# Autodesk Inventor assembly: 0008-10-03 YAxis
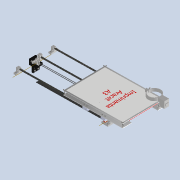
[picture p0: Inventor's stored thumbnail of the model, 180x180]
Saved by Autodesk Inventor 2020 (Build 240168000, 168)
## iProperties
Created: 2021-02-20
Part Number: 0008-10-03 YAxis
Document SubType Name: Assembly
Designer: Iulian Bors
Description: Y axis
Author: Iulian Bors
Subject: 10-03
## Documents named in this file (39)
- Z:\I.A.B\Proiecte\0008 I.A.B 3D 2.1 Imprimanta aracet Metal\10 Mecanic\0008-10-03 YAxis.iam
- Z:\I.A.B\Proiecte\0008 I.A.B 3D 2.1 Imprimanta aracet Metal\10 Mecanic\Foaie A3.ipt
- Z:\I.A.B\Proiecte\0008 I.A.B 3D 2.1 Imprimanta aracet Metal\10 Mecanic\0008-10-1001 NEMA17 - Motor de passo.ipt
- Z:\I.A.B\Proiecte\0008 I.A.B 3D 2.1 Imprimanta aracet Metal\10 Mecanic\0008-10-1011 GT2 Timing Pulley 20 Tooth.ipt
- Z:\I.A.B\Proiecte\0008 I.A.B 3D 2.1 Imprimanta aracet Metal\10 Mecanic\0008-10-1012 16T W6 B3 Without T_Shrinkwrap_1.ipt
- Z:\I.A.B\Proiecte\0008 I.A.B 3D 2.1 Imprimanta aracet Metal\10 Mecanic\0008-10-017 Heated bed.ipt
- Z:\I.A.B\Proiecte\0008 I.A.B 3D 2.1 Imprimanta aracet Metal\10 Mecanic\0008-10-018 Suport Heated Bed.ipt
- Z:\I.A.B\Proiecte\0008 I.A.B 3D 2.1 Imprimanta aracet Metal\10 Mecanic\0008-10-1016 SC10UU.ipt
- Z:\I.A.B\Proiecte\0008 I.A.B 3D 2.1 Imprimanta aracet Metal\10 Mecanic\0008-10-1017 Bara 10.ipt
- Z:\I.A.B\Proiecte\0008 I.A.B 3D 2.1 Imprimanta aracet Metal\10 Mecanic\0008-10-019 Suport Axa Y.ipt
- Z:\I.A.B\Proiecte\0008 I.A.B 3D 2.1 Imprimanta aracet Metal\10 Mecanic\0008-10-020 Suport Axa Y.ipt
- Z:\I.A.B\Proiecte\0008 I.A.B 3D 2.1 Imprimanta aracet Metal\10 Mecanic\0008-10-037.ipt
- Z:\I.A.B\Proiecte\0008 I.A.B 3D 2.1 Imprimanta aracet Metal\10 Mecanic\0008-10-036.ipt
- Z:\I.A.B\Proiecte\0008 I.A.B 3D 2.1 Imprimanta aracet Metal\20 Electric\0008-20-1003 Switch.ipt
- Z:\I.A.B\Proiecte\0008 I.A.B 3D 2.1 Imprimanta aracet Metal\10 Mecanic\0008-10-047 Suport Rulment Sc si curea.ipt
- Z:\I.A.B\Proiecte\0008 I.A.B 3D 2.1 Imprimanta aracet Metal\10 Mecanic\0008-10-048.ipt
- Z:\I.A.B\Proiecte\0008 I.A.B 3D 2.1 Imprimanta aracet Metal\10 Mecanic\0008-10-052 Suport Axa Y +Senzor.ipt
- Z:\I.A.B\Proiecte\0008 I.A.B 3D 2.1 Imprimanta aracet Metal\10 Mecanic\0008-10-054 Suport doking.ipt
- Z:\I.A.B\Proiecte\0008 I.A.B 3D 2.1 Imprimanta aracet Metal\10 Mecanic\0008-10-2016 DIN 315 - M4.ipt
- Z:\I.A.B\Proiecte\0008 I.A.B 3D 2.1 Imprimanta aracet Metal\10 Mecanic\0008-10-2017 DIN 7991 - M4x20.ipt
- Z:\I.A.B\Proiecte\0008 I.A.B 3D 2.1 Imprimanta aracet Metal\10 Mecanic\0008-10-055 Doking.ipt
- Z:\I.A.B\Proiecte\0008 I.A.B 3D 2.1 Imprimanta aracet Metal\10 Mecanic\0008-10-2000 DIN 6912 - M4 x 25.ipt
- Z:\I.A.B\Proiecte\0008 I.A.B 3D 2.1 Imprimanta aracet Metal\20 Electric\0008-20-1007 HEATING BED.ipt
- Z:\I.A.B\Proiecte\0008 I.A.B 3D 2.1 Imprimanta aracet Metal\10 Mecanic\0008-10-01 Sckeleton_Shrinkwrap.ipt
- Z:\I.A.B\Proiecte\0008 I.A.B 3D 2.1 Imprimanta aracet Metal\10 Mecanic\0008-10-2002 DIN 125 - A 4.3.ipt
- Z:\I.A.B\Proiecte\0008 I.A.B 3D 2.1 Imprimanta aracet Metal\10 Mecanic\0008-10-2010 M 5 Canal.ipt
- Z:\I.A.B\Proiecte\0008 I.A.B 3D 2.1 Imprimanta aracet Metal\10 Mecanic\0008-10-2011 DIN 7984 - M5 x 16.ipt
- Z:\I.A.B\Proiecte\0008 I.A.B 3D 2.1 Imprimanta aracet Metal\10 Mecanic\0008-10-2012 DIN 125 - A 5.3.ipt
- Z:\I.A.B\Proiecte\0008 I.A.B 3D 2.1 Imprimanta aracet Metal\10 Mecanic\SurubM4x25.iam
- Z:\I.A.B\Proiecte\0008 I.A.B 3D 2.1 Imprimanta aracet Metal\10 Mecanic\0008-10-2005 DIN 125 - A 3.2.ipt
- Z:\I.A.B\Proiecte\0008 I.A.B 3D 2.1 Imprimanta aracet Metal\10 Mecanic\0008-10-2006 DIN 7984 - M3 x 16.ipt
- Z:\I.A.B\Proiecte\0008 I.A.B 3D 2.1 Imprimanta aracet Metal\10 Mecanic\0008-10-2018 DIN 912 - M4 x 0.7 x 40.ipt
- Z:\I.A.B\Proiecte\0008 I.A.B 3D 2.1 Imprimanta aracet Metal\10 Mecanic\0008-10-2001 DIN 934 - M4 x 0.7.ipt
- Z:\I.A.B\Proiecte\0008 I.A.B 3D 2.1 Imprimanta aracet Metal\10 Mecanic\0008-10-1023 Compress Spring11.ipt
- Z:\I.A.B\Proiecte\0008 I.A.B 3D 2.1 Imprimanta aracet Metal\10 Mecanic\0008-10-03 YAxis\Design Accelerator\Synchronous Belts Transmission1.iam
- Z:\I.A.B\Proiecte\0008 I.A.B 3D 2.1 Imprimanta aracet Metal\10 Mecanic\0008-10-1026 wire chain Y.ipt
- Z:\I.A.B\Proiecte\0008 I.A.B 3D 2.1 Imprimanta aracet Metal\10 Mecanic\0008-10-2024 DIN 7991 - M4  x  35.ipt
- Z:\I.A.B\Proiecte\0008 I.A.B 3D 2.1 Imprimanta aracet Metal\10 Mecanic\0008-10-2027 DIN 7984 - M3 x 5.ipt
- Z:\I.A.B\Proiecte\0008 I.A.B 3D 2.1 Imprimanta aracet Metal\10 Mecanic\0008-10-2040 DIN 7984 - M5 x 20.ipt
## Components (189 placed, 39 different names)
1. Foaie A3.ipt:1 — Mate:59, Flush:56, Flush:57, Angle:8, Mate:216
2. 0008-10-017 Heated bed.ipt:2 — Mate:59, Flush:56, Flush:57, Mate:60, Mate:61, Mate:62, Mate:213, Mate:214, Flush:141
3. 0008-10-018 Suport Heated Bed.ipt:3 — Mate:60, Mate:61, Mate:62, Mate:65, Flush:59, Mate:66, Flush:61, Mate:68, Mate:69, Flush:64, Flush:65, Angle:9, Mate:73, Mate:74, Mate:78, Mate:197, Insert:33, Insert:36, Angle:32, Insert:48, Insert:49, Insert:50, Insert:51, Insert:56, Insert:57, Insert:58, Insert:59, Insert:64, Insert:65, Insert:66, Insert:67, Insert:72, Insert:73, Insert:74, Insert:75, Insert:80, Insert:81, Insert:82, Insert:83, Insert:102, Insert:103, Insert:160, Insert:164, Insert:165, Insert:166, Mate:226, Insert:191
4. 0008-10-1016 SC10UU.ipt:4 — Mate:69, Flush:63, Flush:64, Mate:228
5. 0008-10-1016 SC10UU.ipt:5 — Mate:66, Mate:67, Flush:60, Flush:63
6. 0008-10-1016 SC10UU.ipt:6 — Mate:68, Flush:62, Flush:65, Mate:70
7. 0008-10-1016 SC10UU.ipt:7 — Mate:65, Flush:59, Mate:67, Flush:60, Flush:61, Flush:62, Mate:77
8. 0008-10-1017 Bara 10.ipt:8 — Mate:70, Mate:71, Flush:66, Flush:67, Mate:72
9. 0008-10-020 Suport Axa Y.ipt:9 — Mate:71, Flush:66, Angle:9, Angle:10, Flush:70, Flush:71, Flush:73, Flush:74, Flush:143, Insert:100, Insert:101, Insert:184
10. 0008-10-052 Suport Axa Y +Senzor.ipt:10 — Angle:10, Flush:67, Mate:72, Flush:75, Mate:208, Flush:138, Insert:112, Insert:113, Insert:186
11. 0008-10-1016 SC10UU.ipt:11 — Mate:73, Mate:74, Mate:78, Mate:79, Mate:198, Mate:199
12. 0008-10-1017 Bara 10.ipt:12 — Mate:77, Flush:72
13. 0008-10-020 Suport Axa Y.ipt:13 — Flush:70, Flush:71, Mate:217, Flush:142, Insert:86, Insert:93, Insert:183
14. 0008-10-020 Suport Axa Y.ipt:14 — Angle:12, Insert:132, Insert:133, Insert:185
15. 0008-10-1017 Bara 10.ipt:15 — Mate:79, Flush:72, Mate:80, Mate:81
16. 0008-10-019 Suport Axa Y.ipt:16 — Mate:80, Flush:73, Flush:74, Angle:27, Mate:182, Insert:94, Insert:95, Insert:187
17. 0008-10-019 Suport Axa Y.ipt:17 — Mate:81, Flush:75, Angle:12, Insert:114, Insert:115, Insert:188
18. 0008-10-1001 NEMA17 - Motor de passo.ipt:18 — Mate:201, Insert:43, Mate:218
19. 0008-10-1011 GT2 Timing Pulley 20 Tooth.ipt:19 — Flush:120
20. 0008-10-037.ipt:20 — Mate:181, Mate:182, Mate:184, Insert:124, Insert:125, Insert:126, Insert:127, Insert:151, Insert:158, Mate:221
21. 0008-10-036.ipt:21 — Insert:22, Angle:27, Mate:181, Mate:184, Insert:190
22. 0008-10-1012 16T W6 B3 Without T_Shrinkwrap_1.ipt:22 — Insert:22, Flush:120
23. 0008-10-047 Suport Rulment Sc si curea.ipt:23 — Mate:197, Mate:198, Mate:199
24. 0008-10-048.ipt:24 — Mate:201, Insert:43, Mate:218, Insert:138, Insert:139, Insert:140, Insert:141, Insert:144, Insert:147
25. 0008-20-1003 Switch.ipt:25 — Mate:208, Flush:138
26. 0008-10-054 Suport doking.ipt:26 — Flush:139, Mate:211, Mate:212, Insert:39, Insert:191, Mate:229
27. 0008-10-055 Doking.ipt:32 — Flush:139, Angle:32, Mate:211, Mate:212, Insert:42
28. 0008-20-1007 HEATING BED.ipt:35 — Mate:214, Mate:215, Flush:140, Mate:216, Insert:168, Insert:176, Insert:177, Insert:178
29. 0008-20-1007 HEATING BED.ipt:36 — Mate:213, Mate:215, Flush:140, Flush:141, Insert:179, Insert:180, Insert:181, Insert:182
30. 0008-10-01 Sckeleton_Shrinkwrap.ipt:37 — Mate:217, Flush:142, Flush:143, Mate:223, Mate:225
31. Synchronous Belts Transmission1.iam:162 [sub-assembly]
32. SurubM4x25:3 [sub-assembly] — Insert:183
33. SurubM4x25:4 [sub-assembly] — Insert:184
34. SurubM4x25:5 [sub-assembly] — Insert:185
35. SurubM4x25:6 [sub-assembly] — Insert:186
36. SurubM4x25:7 [sub-assembly] — Insert:187
37. SurubM4x25:8 [sub-assembly] — Insert:188
38. DIN 7984 M5 x 20:1 — Insert:190
39. 0008-10-2027 DIN 7984 - M3 x 5.ipt:167 — Insert:167
40. 0008-10-2005 DIN 125 - A 3.2.ipt:168 — Insert:167, Insert:168
41. 0008-10-2027 DIN 7984 - M3 x 5.ipt:169
42. 0008-10-2005 DIN 125 - A 3.2.ipt:170 — Insert:176
43. 0008-10-2027 DIN 7984 - M3 x 5.ipt:171
44. 0008-10-2005 DIN 125 - A 3.2.ipt:172 — Insert:177
45. 0008-10-2027 DIN 7984 - M3 x 5.ipt:173
46. 0008-10-2005 DIN 125 - A 3.2.ipt:174 — Insert:178
47. 0008-10-2027 DIN 7984 - M3 x 5.ipt:175
48. 0008-10-2005 DIN 125 - A 3.2.ipt:176 — Insert:182
49. 0008-10-2027 DIN 7984 - M3 x 5.ipt:177
50. 0008-10-2005 DIN 125 - A 3.2.ipt:178 — Insert:181
51. 0008-10-2027 DIN 7984 - M3 x 5.ipt:179
52. 0008-10-2005 DIN 125 - A 3.2.ipt:180 — Insert:180
53. 0008-10-2027 DIN 7984 - M3 x 5.ipt:181
54. 0008-10-2005 DIN 125 - A 3.2.ipt:182 — Insert:179
55. 0008-10-2016 DIN 315 - M4.ipt:38 — Insert:159
56. 0008-10-2024 DIN 7991 - M4  x  35.ipt:39 — Insert:159, Insert:160
57. 0008-10-2016 DIN 315 - M4.ipt:40
58. 0008-10-2024 DIN 7991 - M4  x  35.ipt:41 — Insert:164, Mate:227
59. 0008-10-2016 DIN 315 - M4.ipt:42
60. 0008-10-1026 wire chain Y.ipt:43 — Mate:223, Mate:225, Mate:228
61. 0008-10-2024 DIN 7991 - M4  x  35.ipt:44 — Insert:165
62. 0008-10-2016 DIN 315 - M4.ipt:45
63. 0008-10-2024 DIN 7991 - M4  x  35.ipt:46 — Insert:166
64. 0008-10-2010 M 5 Canal.ipt:47
65. 0008-10-2011 DIN 7984 - M5 x 16.ipt:48
66. 0008-10-2012 DIN 125 - A 5.3.ipt:49 — Insert:93
67. 0008-10-2010 M 5 Canal.ipt:50
68. 0008-10-2011 DIN 7984 - M5 x 16.ipt:51
69. 0008-10-2012 DIN 125 - A 5.3.ipt:52 — Insert:94
70. 0008-10-2010 M 5 Canal.ipt:53
71. 0008-10-2011 DIN 7984 - M5 x 16.ipt:54
72. 0008-10-2012 DIN 125 - A 5.3.ipt:55 — Insert:95
73. 0008-10-2010 M 5 Canal.ipt:56
74. 0008-10-2011 DIN 7984 - M5 x 16.ipt:57
75. 0008-10-2012 DIN 125 - A 5.3.ipt:58 — Insert:101
76. 0008-10-2010 M 5 Canal.ipt:59
77. 0008-10-2011 DIN 7984 - M5 x 16.ipt:60
78. 0008-10-2012 DIN 125 - A 5.3.ipt:61 — Insert:100
79. SurubM4x25.iam:62 [sub-assembly] — Insert:102
80. SurubM4x25.iam:63 [sub-assembly] — Insert:103
81. 0008-10-2010 M 5 Canal.ipt:64
82. 0008-10-2011 DIN 7984 - M5 x 16.ipt:65
83. 0008-10-2012 DIN 125 - A 5.3.ipt:66 — Insert:112
84. 0008-10-2010 M 5 Canal.ipt:67
85. 0008-10-2011 DIN 7984 - M5 x 16.ipt:68
86. 0008-10-2012 DIN 125 - A 5.3.ipt:69 — Insert:113
87. 0008-10-2010 M 5 Canal.ipt:70
88. 0008-10-2011 DIN 7984 - M5 x 16.ipt:71
89. 0008-10-2012 DIN 125 - A 5.3.ipt:72 — Insert:114
90. 0008-10-2010 M 5 Canal.ipt:73
91. 0008-10-2011 DIN 7984 - M5 x 16.ipt:74
92. 0008-10-2012 DIN 125 - A 5.3.ipt:75 — Insert:115
93. 0008-10-2010 M 5 Canal.ipt:76
94. 0008-10-2011 DIN 7984 - M5 x 16.ipt:77
95. 0008-10-2012 DIN 125 - A 5.3.ipt:78 — Insert:125
96. 0008-10-2010 M 5 Canal.ipt:79
97. 0008-10-2011 DIN 7984 - M5 x 16.ipt:80
98. 0008-10-2012 DIN 125 - A 5.3.ipt:81 — Insert:126
99. 0008-10-2010 M 5 Canal.ipt:82
100. 0008-10-2011 DIN 7984 - M5 x 16.ipt:83
101. 0008-10-2012 DIN 125 - A 5.3.ipt:84 — Insert:127
102. 0008-10-2010 M 5 Canal.ipt:85
103. 0008-10-2011 DIN 7984 - M5 x 16.ipt:86
104. 0008-10-2012 DIN 125 - A 5.3.ipt:87 — Insert:124
105. 0008-10-2010 M 5 Canal.ipt:88
106. 0008-10-2011 DIN 7984 - M5 x 16.ipt:89
107. 0008-10-2012 DIN 125 - A 5.3.ipt:90 — Insert:132
108. 0008-10-2010 M 5 Canal.ipt:91
109. 0008-10-2011 DIN 7984 - M5 x 16.ipt:92
110. 0008-10-2012 DIN 125 - A 5.3.ipt:93 — Insert:133
111. 0008-10-2005 DIN 125 - A 3.2.ipt:94 — Insert:134, Insert:141
112. 0008-10-2006 DIN 7984 - M3 x 16.ipt:95 — Insert:134
113. 0008-10-2005 DIN 125 - A 3.2.ipt:96 — Insert:139
114. 0008-10-2006 DIN 7984 - M3 x 16.ipt:97
115. 0008-10-2005 DIN 125 - A 3.2.ipt:98 — Insert:138
116. 0008-10-2006 DIN 7984 - M3 x 16.ipt:99
117. 0008-10-2005 DIN 125 - A 3.2.ipt:100 — Insert:140
118. 0008-10-2006 DIN 7984 - M3 x 16.ipt:101
119. 0008-10-2000 DIN 6912 - M4 x 25.ipt:102 — Insert:142, Insert:143
120. 0008-10-2012 DIN 125 - A 5.3.ipt:103 — Insert:142, Insert:144
121. 0008-10-2010 M 5 Canal.ipt:104 — Insert:143
122. 0008-10-2000 DIN 6912 - M4 x 25.ipt:105
123. 0008-10-2012 DIN 125 - A 5.3.ipt:106 — Insert:147
124. 0008-10-2010 M 5 Canal.ipt:107
125. 0008-10-2018 DIN 912 - M4 x 0.7 x 40.ipt:108
126. 0008-10-2002 DIN 125 - A 4.3.ipt:109
127. 0008-10-2001 DIN 934 - M4 x 0.7.ipt:110
128. 0008-10-2002 DIN 125 - A 4.3.ipt:111 — Insert:151
129. 0008-10-2018 DIN 912 - M4 x 0.7 x 40.ipt:112 — Mate:222
130. 0008-10-2002 DIN 125 - A 4.3.ipt:113
131. 0008-10-2001 DIN 934 - M4 x 0.7.ipt:114
132. 0008-10-2002 DIN 125 - A 4.3.ipt:115 — Insert:158
133. 0008-10-2000 DIN 6912 - M4 x 25.ipt:116
134. 0008-10-2002 DIN 125 - A 4.3.ipt:117 — Insert:48
135. 0008-10-2000 DIN 6912 - M4 x 25.ipt:118
136. 0008-10-2002 DIN 125 - A 4.3.ipt:119 — Insert:49
137. 0008-10-2000 DIN 6912 - M4 x 25.ipt:120
138. 0008-10-2002 DIN 125 - A 4.3.ipt:121 — Insert:50
139. 0008-10-2000 DIN 6912 - M4 x 25.ipt:122
140. 0008-10-2002 DIN 125 - A 4.3.ipt:123 — Insert:51
141. 0008-10-2000 DIN 6912 - M4 x 25.ipt:124
142. 0008-10-2002 DIN 125 - A 4.3.ipt:125 — Insert:56
143. 0008-10-2000 DIN 6912 - M4 x 25.ipt:126
144. 0008-10-2002 DIN 125 - A 4.3.ipt:127 — Insert:59
145. 0008-10-2000 DIN 6912 - M4 x 25.ipt:128
146. 0008-10-2002 DIN 125 - A 4.3.ipt:129 — Insert:58
147. 0008-10-2000 DIN 6912 - M4 x 25.ipt:130
148. 0008-10-2002 DIN 125 - A 4.3.ipt:131 — Insert:57
149. 0008-10-2000 DIN 6912 - M4 x 25.ipt:132
150. 0008-10-2002 DIN 125 - A 4.3.ipt:133 — Insert:64
151. 0008-10-2000 DIN 6912 - M4 x 25.ipt:134
152. 0008-10-2002 DIN 125 - A 4.3.ipt:135 — Insert:65
153. 0008-10-2000 DIN 6912 - M4 x 25.ipt:136
154. 0008-10-2002 DIN 125 - A 4.3.ipt:137 — Insert:66
155. 0008-10-2000 DIN 6912 - M4 x 25.ipt:138
156. 0008-10-2002 DIN 125 - A 4.3.ipt:139 — Insert:67
157. 0008-10-2000 DIN 6912 - M4 x 25.ipt:140
158. 0008-10-2002 DIN 125 - A 4.3.ipt:141 — Insert:72
159. 0008-10-2000 DIN 6912 - M4 x 25.ipt:142
160. 0008-10-2002 DIN 125 - A 4.3.ipt:143 — Insert:74
161. 0008-10-2000 DIN 6912 - M4 x 25.ipt:144
162. 0008-10-2002 DIN 125 - A 4.3.ipt:145 — Insert:75
163. 0008-10-2000 DIN 6912 - M4 x 25.ipt:146
164. 0008-10-2002 DIN 125 - A 4.3.ipt:147 — Insert:73
165. 0008-10-2000 DIN 6912 - M4 x 25.ipt:148
166. 0008-10-2002 DIN 125 - A 4.3.ipt:149 — Insert:81
167. 0008-10-2000 DIN 6912 - M4 x 25.ipt:150
168. 0008-10-2002 DIN 125 - A 4.3.ipt:151 — Insert:83
169. 0008-10-2000 DIN 6912 - M4 x 25.ipt:152
170. 0008-10-2002 DIN 125 - A 4.3.ipt:153 — Insert:82
171. 0008-10-2000 DIN 6912 - M4 x 25.ipt:154
172. 0008-10-2002 DIN 125 - A 4.3.ipt:155 — Insert:80
173. 0008-10-2010 M 5 Canal.ipt:156
174. 0008-10-2011 DIN 7984 - M5 x 16.ipt:157
175. 0008-10-2012 DIN 125 - A 5.3.ipt:158 — Insert:86
176. 0008-10-2016 DIN 315 - M4.ipt:27 — Insert:34
177. 0008-10-2017 DIN 7991 - M4x20.ipt:28 — Insert:33, Insert:34
178. 0008-10-2016 DIN 315 - M4.ipt:29
179. 0008-10-2017 DIN 7991 - M4x20.ipt:30 — Insert:36, Mate:229
180. 0008-10-2016 DIN 315 - M4.ipt:31 — Insert:40
181. 0008-10-2000 DIN 6912 - M4 x 25.ipt:33 — Insert:39, Insert:40
182. 0008-10-2016 DIN 315 - M4.ipt:34
183. 0008-10-2000 DIN 6912 - M4 x 25.ipt:159 — Insert:42
184. 0008-10-1023 Compress Spring11.ipt:160 — Mate:221, Mate:222
185. 0008-10-1023 Compress Spring11.ipt:161
186. 0008-10-1023 Compress Spring11.ipt:163 — Mate:226, Mate:227
187. 0008-10-1023 Compress Spring11.ipt:164
188. 0008-10-1023 Compress Spring11.ipt:165
189. 0008-10-1023 Compress Spring11.ipt:166
## Component patterns: (2 elements, first: 0008-10-1023 Compress Spring11.ipt:160), (4 elements, first: 0008-10-1023 Compress Spring11.ipt:163)
## Relationships (233: Insert 155, Mate 45, Flush 26, Angle 7)
- Mate:59: Foaie A3.ipt:1 ↔ 0008-10-017 Heated bed.ipt:2
- Flush:56 (-10 mm): Foaie A3.ipt:1 ↔ 0008-10-017 Heated bed.ipt:2
- Flush:57 (-10 mm): Foaie A3.ipt:1 ↔ 0008-10-017 Heated bed.ipt:2
- Mate:60 (25 mm): 0008-10-017 Heated bed.ipt:2 ↔ 0008-10-018 Suport Heated Bed.ipt:3
- Mate:61: 0008-10-017 Heated bed.ipt:2 ↔ 0008-10-018 Suport Heated Bed.ipt:3
- Mate:62: 0008-10-017 Heated bed.ipt:2 ↔ 0008-10-018 Suport Heated Bed.ipt:3
- Angle:8 (0 deg): Foaie A3.ipt:1
- Mate:65: 0008-10-018 Suport Heated Bed.ipt:3 ↔ 0008-10-1016 SC10UU.ipt:7
- Flush:59 (5 mm): 0008-10-018 Suport Heated Bed.ipt:3 ↔ 0008-10-1016 SC10UU.ipt:7
- Mate:66: 0008-10-018 Suport Heated Bed.ipt:3 ↔ 0008-10-1016 SC10UU.ipt:5
- Mate:67 (100 mm): 0008-10-1016 SC10UU.ipt:5 ↔ 0008-10-1016 SC10UU.ipt:7
- Flush:60: 0008-10-1016 SC10UU.ipt:5 ↔ 0008-10-1016 SC10UU.ipt:7
- Flush:61 (135 mm): 0008-10-018 Suport Heated Bed.ipt:3 ↔ 0008-10-1016 SC10UU.ipt:7
- Mate:68: 0008-10-018 Suport Heated Bed.ipt:3 ↔ 0008-10-1016 SC10UU.ipt:6
- Flush:62: 0008-10-1016 SC10UU.ipt:6 ↔ 0008-10-1016 SC10UU.ipt:7
- Mate:69: 0008-10-018 Suport Heated Bed.ipt:3 ↔ 0008-10-1016 SC10UU.ipt:4
- Flush:63: 0008-10-1016 SC10UU.ipt:4 ↔ 0008-10-1016 SC10UU.ipt:5
- Flush:64 (5 mm): 0008-10-018 Suport Heated Bed.ipt:3 ↔ 0008-10-1016 SC10UU.ipt:4
- Flush:65 (5 mm): 0008-10-018 Suport Heated Bed.ipt:3 ↔ 0008-10-1016 SC10UU.ipt:6
- Mate:70: 0008-10-1016 SC10UU.ipt:6 ↔ 0008-10-1017 Bara 10.ipt:8
- Mate:71: 0008-10-1017 Bara 10.ipt:8 ↔ 0008-10-020 Suport Axa Y.ipt:9
- Flush:66: 0008-10-1017 Bara 10.ipt:8 ↔ 0008-10-020 Suport Axa Y.ipt:9
- Angle:9 (0 deg): 0008-10-018 Suport Heated Bed.ipt:3 ↔ 0008-10-020 Suport Axa Y.ipt:9
- Angle:10 (0 deg): 0008-10-020 Suport Axa Y.ipt:9 ↔ 0008-10-052 Suport Axa Y +Senzor.ipt:10
- Flush:67: 0008-10-1017 Bara 10.ipt:8 ↔ 0008-10-052 Suport Axa Y +Senzor.ipt:10
- Mate:72: 0008-10-1017 Bara 10.ipt:8 ↔ 0008-10-052 Suport Axa Y +Senzor.ipt:10
- Mate:73 (5 mm): 0008-10-018 Suport Heated Bed.ipt:3 ↔ 0008-10-1016 SC10UU.ipt:11
- Mate:74 (30 mm): 0008-10-018 Suport Heated Bed.ipt:3 ↔ 0008-10-1016 SC10UU.ipt:11
- [Mate]: 0008-10-1017 Bara 10.ipt:12 ↔ 0008-10-020 Suport Axa Y.ipt:13
- [Flush]: 0008-10-1017 Bara 10.ipt:12 ↔ 0008-10-020 Suport Axa Y.ipt:13
- [Angle] (0 deg): 0008-10-020 Suport Axa Y.ipt:13 ↔ 0008-10-020 Suport Axa Y.ipt:14
- [Flush]: 0008-10-1017 Bara 10.ipt:12 ↔ 0008-10-020 Suport Axa Y.ipt:14
- [Mate]: 0008-10-1017 Bara 10.ipt:12 ↔ 0008-10-020 Suport Axa Y.ipt:14
- Mate:77: 0008-10-1016 SC10UU.ipt:7 ↔ 0008-10-1017 Bara 10.ipt:12
- Mate:78 (-17.5 mm): 0008-10-018 Suport Heated Bed.ipt:3 ↔ 0008-10-1016 SC10UU.ipt:11
- Flush:70: 0008-10-020 Suport Axa Y.ipt:9 ↔ 0008-10-020 Suport Axa Y.ipt:13
- Flush:71: 0008-10-020 Suport Axa Y.ipt:9 ↔ 0008-10-020 Suport Axa Y.ipt:13
- Mate:79: 0008-10-1016 SC10UU.ipt:11 ↔ 0008-10-1017 Bara 10.ipt:15
- Flush:72: 0008-10-1017 Bara 10.ipt:12 ↔ 0008-10-1017 Bara 10.ipt:15
- Mate:80: 0008-10-1017 Bara 10.ipt:15 ↔ 0008-10-019 Suport Axa Y.ipt:16
- Flush:73: 0008-10-020 Suport Axa Y.ipt:9 ↔ 0008-10-019 Suport Axa Y.ipt:16
- Flush:74: 0008-10-020 Suport Axa Y.ipt:9 ↔ 0008-10-019 Suport Axa Y.ipt:16
- Mate:81: 0008-10-1017 Bara 10.ipt:15 ↔ 0008-10-019 Suport Axa Y.ipt:17
- Flush:75: 0008-10-052 Suport Axa Y +Senzor.ipt:10 ↔ 0008-10-019 Suport Axa Y.ipt:17
- Angle:12 (0 deg): 0008-10-020 Suport Axa Y.ipt:14 ↔ 0008-10-019 Suport Axa Y.ipt:17
- [Insert]: 0008-10-1001 NEMA17 - Motor de passo.ipt:18 ↔ 0008-10-1011 GT2 Timing Pulley 20 Tooth.ipt:19
- Insert:22 (0.8 mm): 0008-10-036.ipt:21 ↔ 0008-10-1012 16T W6 B3 Without T_Shrinkwrap_1.ipt:22
- Flush:120: 0008-10-1011 GT2 Timing Pulley 20 Tooth.ipt:19 ↔ 0008-10-1012 16T W6 B3 Without T_Shrinkwrap_1.ipt:22
- Angle:27 (0 deg): 0008-10-019 Suport Axa Y.ipt:16 ↔ 0008-10-036.ipt:21
- Mate:181 (0.5 mm): 0008-10-037.ipt:20 ↔ 0008-10-036.ipt:21
- Mate:182: 0008-10-019 Suport Axa Y.ipt:16 ↔ 0008-10-037.ipt:20
- Mate:184 (0.5 mm): 0008-10-037.ipt:20 ↔ 0008-10-036.ipt:21
- Mate:197: 0008-10-018 Suport Heated Bed.ipt:3 ↔ 0008-10-047 Suport Rulment Sc si curea.ipt:23
- Mate:198: 0008-10-1016 SC10UU.ipt:11 ↔ 0008-10-047 Suport Rulment Sc si curea.ipt:23
- Mate:199: 0008-10-1016 SC10UU.ipt:11 ↔ 0008-10-047 Suport Rulment Sc si curea.ipt:23
- Mate:201: 0008-10-1001 NEMA17 - Motor de passo.ipt:18 ↔ 0008-10-048.ipt:24
- Mate:208: 0008-10-052 Suport Axa Y +Senzor.ipt:10 ↔ 0008-20-1003 Switch.ipt:25
- Flush:138 (5 mm): 0008-10-052 Suport Axa Y +Senzor.ipt:10 ↔ 0008-20-1003 Switch.ipt:25
- Insert:33: 0008-10-018 Suport Heated Bed.ipt:3 ↔ 0008-10-2017 DIN 7991 - M4x20.ipt:28
- Insert:34: 0008-10-2016 DIN 315 - M4.ipt:27 ↔ 0008-10-2017 DIN 7991 - M4x20.ipt:28
- [Insert]: 0008-10-2016 DIN 315 - M4.ipt:29 ↔ 0008-10-2017 DIN 7991 - M4x20.ipt:30
- Insert:36: 0008-10-018 Suport Heated Bed.ipt:3 ↔ 0008-10-2017 DIN 7991 - M4x20.ipt:30
- Flush:139: 0008-10-054 Suport doking.ipt:26 ↔ 0008-10-055 Doking.ipt:32
- Angle:32 (0 deg): 0008-10-018 Suport Heated Bed.ipt:3 ↔ 0008-10-055 Doking.ipt:32
- Mate:211: 0008-10-054 Suport doking.ipt:26 ↔ 0008-10-055 Doking.ipt:32
- Mate:212: 0008-10-054 Suport doking.ipt:26 ↔ 0008-10-055 Doking.ipt:32
- Insert:39: 0008-10-054 Suport doking.ipt:26 ↔ 0008-10-2000 DIN 6912 - M4 x 25.ipt:33
- Insert:40 (-3 mm): 0008-10-2016 DIN 315 - M4.ipt:31 ↔ 0008-10-2000 DIN 6912 - M4 x 25.ipt:33
- Mate:213: 0008-10-017 Heated bed.ipt:2 ↔ 0008-20-1007 HEATING BED.ipt:36
- Mate:214: 0008-10-017 Heated bed.ipt:2 ↔ 0008-20-1007 HEATING BED.ipt:35
- Mate:215 (6 mm): 0008-20-1007 HEATING BED.ipt:35 ↔ 0008-20-1007 HEATING BED.ipt:36
- Flush:140: 0008-20-1007 HEATING BED.ipt:35 ↔ 0008-20-1007 HEATING BED.ipt:36
- Mate:216: Foaie A3.ipt:1 ↔ 0008-20-1007 HEATING BED.ipt:35
- Flush:141: 0008-10-017 Heated bed.ipt:2 ↔ 0008-20-1007 HEATING BED.ipt:36
- Mate:217: 0008-10-020 Suport Axa Y.ipt:13 ↔ 0008-10-01 Sckeleton_Shrinkwrap.ipt:37
- Flush:142: 0008-10-020 Suport Axa Y.ipt:13 ↔ 0008-10-01 Sckeleton_Shrinkwrap.ipt:37
- Flush:143 (193.5 mm): 0008-10-020 Suport Axa Y.ipt:9 ↔ 0008-10-01 Sckeleton_Shrinkwrap.ipt:37
- [Insert] (-3 mm): 0008-10-2016 DIN 315 - M4.ipt:34 ↔ 0008-10-2000 DIN 6912 - M4 x 25.ipt:159
- Insert:42 (1 mm): 0008-10-055 Doking.ipt:32 ↔ 0008-10-2000 DIN 6912 - M4 x 25.ipt:159
- Insert:43: 0008-10-1001 NEMA17 - Motor de passo.ipt:18 ↔ 0008-10-048.ipt:24
- Mate:218: 0008-10-1001 NEMA17 - Motor de passo.ipt:18 ↔ 0008-10-048.ipt:24
- [Insert]: 0008-10-2000 DIN 6912 - M4 x 25.ipt:116 ↔ 0008-10-2002 DIN 125 - A 4.3.ipt:117
- [Insert]: 0008-10-2000 DIN 6912 - M4 x 25.ipt:118 ↔ 0008-10-2002 DIN 125 - A 4.3.ipt:119
- [Insert]: 0008-10-2000 DIN 6912 - M4 x 25.ipt:120 ↔ 0008-10-2002 DIN 125 - A 4.3.ipt:121
- [Insert]: 0008-10-2000 DIN 6912 - M4 x 25.ipt:122 ↔ 0008-10-2002 DIN 125 - A 4.3.ipt:123
- Insert:48: 0008-10-018 Suport Heated Bed.ipt:3 ↔ 0008-10-2002 DIN 125 - A 4.3.ipt:117
- Insert:49: 0008-10-018 Suport Heated Bed.ipt:3 ↔ 0008-10-2002 DIN 125 - A 4.3.ipt:119
- Insert:50: 0008-10-018 Suport Heated Bed.ipt:3 ↔ 0008-10-2002 DIN 125 - A 4.3.ipt:121
- Insert:51: 0008-10-018 Suport Heated Bed.ipt:3 ↔ 0008-10-2002 DIN 125 - A 4.3.ipt:123
- [Insert]: 0008-10-2000 DIN 6912 - M4 x 25.ipt:124 ↔ 0008-10-2002 DIN 125 - A 4.3.ipt:125
- [Insert]: 0008-10-2000 DIN 6912 - M4 x 25.ipt:126 ↔ 0008-10-2002 DIN 125 - A 4.3.ipt:127
- [Insert]: 0008-10-2000 DIN 6912 - M4 x 25.ipt:128 ↔ 0008-10-2002 DIN 125 - A 4.3.ipt:129
- [Insert]: 0008-10-2000 DIN 6912 - M4 x 25.ipt:130 ↔ 0008-10-2002 DIN 125 - A 4.3.ipt:131
- Insert:56: 0008-10-018 Suport Heated Bed.ipt:3 ↔ 0008-10-2002 DIN 125 - A 4.3.ipt:125
- Insert:57: 0008-10-018 Suport Heated Bed.ipt:3 ↔ 0008-10-2002 DIN 125 - A 4.3.ipt:131
- Insert:58: 0008-10-018 Suport Heated Bed.ipt:3 ↔ 0008-10-2002 DIN 125 - A 4.3.ipt:129
- Insert:59: 0008-10-018 Suport Heated Bed.ipt:3 ↔ 0008-10-2002 DIN 125 - A 4.3.ipt:127
- [Insert]: 0008-10-2000 DIN 6912 - M4 x 25.ipt:132 ↔ 0008-10-2002 DIN 125 - A 4.3.ipt:133
- [Insert]: 0008-10-2000 DIN 6912 - M4 x 25.ipt:134 ↔ 0008-10-2002 DIN 125 - A 4.3.ipt:135
- [Insert]: 0008-10-2000 DIN 6912 - M4 x 25.ipt:136 ↔ 0008-10-2002 DIN 125 - A 4.3.ipt:137
- [Insert]: 0008-10-2000 DIN 6912 - M4 x 25.ipt:138 ↔ 0008-10-2002 DIN 125 - A 4.3.ipt:139
- Insert:64: 0008-10-018 Suport Heated Bed.ipt:3 ↔ 0008-10-2002 DIN 125 - A 4.3.ipt:133
- Insert:65: 0008-10-018 Suport Heated Bed.ipt:3 ↔ 0008-10-2002 DIN 125 - A 4.3.ipt:135
- Insert:66: 0008-10-018 Suport Heated Bed.ipt:3 ↔ 0008-10-2002 DIN 125 - A 4.3.ipt:137
- Insert:67: 0008-10-018 Suport Heated Bed.ipt:3 ↔ 0008-10-2002 DIN 125 - A 4.3.ipt:139
- [Insert]: 0008-10-2000 DIN 6912 - M4 x 25.ipt:140 ↔ 0008-10-2002 DIN 125 - A 4.3.ipt:141
- [Insert]: 0008-10-2000 DIN 6912 - M4 x 25.ipt:142 ↔ 0008-10-2002 DIN 125 - A 4.3.ipt:143
- [Insert]: 0008-10-2000 DIN 6912 - M4 x 25.ipt:144 ↔ 0008-10-2002 DIN 125 - A 4.3.ipt:145
- [Insert]: 0008-10-2000 DIN 6912 - M4 x 25.ipt:146 ↔ 0008-10-2002 DIN 125 - A 4.3.ipt:147
- Insert:72: 0008-10-018 Suport Heated Bed.ipt:3 ↔ 0008-10-2002 DIN 125 - A 4.3.ipt:141
- Insert:73: 0008-10-018 Suport Heated Bed.ipt:3 ↔ 0008-10-2002 DIN 125 - A 4.3.ipt:147
- Insert:74: 0008-10-018 Suport Heated Bed.ipt:3 ↔ 0008-10-2002 DIN 125 - A 4.3.ipt:143
- Insert:75: 0008-10-018 Suport Heated Bed.ipt:3 ↔ 0008-10-2002 DIN 125 - A 4.3.ipt:145
- [Insert]: 0008-10-2000 DIN 6912 - M4 x 25.ipt:148 ↔ 0008-10-2002 DIN 125 - A 4.3.ipt:149
- [Insert]: 0008-10-2000 DIN 6912 - M4 x 25.ipt:150 ↔ 0008-10-2002 DIN 125 - A 4.3.ipt:151
- [Insert]: 0008-10-2000 DIN 6912 - M4 x 25.ipt:152 ↔ 0008-10-2002 DIN 125 - A 4.3.ipt:153
- [Insert]: 0008-10-2000 DIN 6912 - M4 x 25.ipt:154 ↔ 0008-10-2002 DIN 125 - A 4.3.ipt:155
- Insert:80: 0008-10-018 Suport Heated Bed.ipt:3 ↔ 0008-10-2002 DIN 125 - A 4.3.ipt:155
- Insert:81: 0008-10-018 Suport Heated Bed.ipt:3 ↔ 0008-10-2002 DIN 125 - A 4.3.ipt:149
- Insert:82: 0008-10-018 Suport Heated Bed.ipt:3 ↔ 0008-10-2002 DIN 125 - A 4.3.ipt:153
- Insert:83: 0008-10-018 Suport Heated Bed.ipt:3 ↔ 0008-10-2002 DIN 125 - A 4.3.ipt:151
- [Insert] (-5 mm): 0008-10-2010 M 5 Canal.ipt:156 ↔ 0008-10-2011 DIN 7984 - M5 x 16.ipt:157
- [Insert]: 0008-10-2011 DIN 7984 - M5 x 16.ipt:157 ↔ 0008-10-2012 DIN 125 - A 5.3.ipt:158
- Insert:86: 0008-10-020 Suport Axa Y.ipt:13 ↔ 0008-10-2012 DIN 125 - A 5.3.ipt:158
- [Insert] (-5 mm): 0008-10-2010 M 5 Canal.ipt:47 ↔ 0008-10-2011 DIN 7984 - M5 x 16.ipt:48
- [Insert]: 0008-10-2011 DIN 7984 - M5 x 16.ipt:48 ↔ 0008-10-2012 DIN 125 - A 5.3.ipt:49
- [Insert] (-5 mm): 0008-10-2010 M 5 Canal.ipt:50 ↔ 0008-10-2011 DIN 7984 - M5 x 16.ipt:51
- [Insert]: 0008-10-2011 DIN 7984 - M5 x 16.ipt:51 ↔ 0008-10-2012 DIN 125 - A 5.3.ipt:52
- [Insert] (-5 mm): 0008-10-2010 M 5 Canal.ipt:53 ↔ 0008-10-2011 DIN 7984 - M5 x 16.ipt:54
- [Insert]: 0008-10-2011 DIN 7984 - M5 x 16.ipt:54 ↔ 0008-10-2012 DIN 125 - A 5.3.ipt:55
- Insert:93: 0008-10-020 Suport Axa Y.ipt:13 ↔ 0008-10-2012 DIN 125 - A 5.3.ipt:49
- Insert:94: 0008-10-019 Suport Axa Y.ipt:16 ↔ 0008-10-2012 DIN 125 - A 5.3.ipt:52
- Insert:95: 0008-10-019 Suport Axa Y.ipt:16 ↔ 0008-10-2012 DIN 125 - A 5.3.ipt:55
- [Insert] (-5 mm): 0008-10-2010 M 5 Canal.ipt:56 ↔ 0008-10-2011 DIN 7984 - M5 x 16.ipt:57
- [Insert]: 0008-10-2011 DIN 7984 - M5 x 16.ipt:57 ↔ 0008-10-2012 DIN 125 - A 5.3.ipt:58
- [Insert] (-5 mm): 0008-10-2010 M 5 Canal.ipt:59 ↔ 0008-10-2011 DIN 7984 - M5 x 16.ipt:60
- [Insert]: 0008-10-2011 DIN 7984 - M5 x 16.ipt:60 ↔ 0008-10-2012 DIN 125 - A 5.3.ipt:61
- Insert:100: 0008-10-020 Suport Axa Y.ipt:9 ↔ 0008-10-2012 DIN 125 - A 5.3.ipt:61
- Insert:101: 0008-10-020 Suport Axa Y.ipt:9 ↔ 0008-10-2012 DIN 125 - A 5.3.ipt:58
- Insert:102: 0008-10-018 Suport Heated Bed.ipt:3 ↔ SurubM4x25.iam:62
- Insert:103: 0008-10-018 Suport Heated Bed.ipt:3 ↔ SurubM4x25.iam:63
- [Insert] (-5 mm): 0008-10-2010 M 5 Canal.ipt:64 ↔ 0008-10-2011 DIN 7984 - M5 x 16.ipt:65
- [Insert]: 0008-10-2011 DIN 7984 - M5 x 16.ipt:65 ↔ 0008-10-2012 DIN 125 - A 5.3.ipt:66
- [Insert] (-5 mm): 0008-10-2010 M 5 Canal.ipt:67 ↔ 0008-10-2011 DIN 7984 - M5 x 16.ipt:68
- [Insert]: 0008-10-2011 DIN 7984 - M5 x 16.ipt:68 ↔ 0008-10-2012 DIN 125 - A 5.3.ipt:69
- [Insert] (-5 mm): 0008-10-2010 M 5 Canal.ipt:70 ↔ 0008-10-2011 DIN 7984 - M5 x 16.ipt:71
- [Insert]: 0008-10-2011 DIN 7984 - M5 x 16.ipt:71 ↔ 0008-10-2012 DIN 125 - A 5.3.ipt:72
- [Insert] (-5 mm): 0008-10-2010 M 5 Canal.ipt:73 ↔ 0008-10-2011 DIN 7984 - M5 x 16.ipt:74
- [Insert]: 0008-10-2011 DIN 7984 - M5 x 16.ipt:74 ↔ 0008-10-2012 DIN 125 - A 5.3.ipt:75
- Insert:112: 0008-10-052 Suport Axa Y +Senzor.ipt:10 ↔ 0008-10-2012 DIN 125 - A 5.3.ipt:66
- Insert:113: 0008-10-052 Suport Axa Y +Senzor.ipt:10 ↔ 0008-10-2012 DIN 125 - A 5.3.ipt:69
- Insert:114: 0008-10-019 Suport Axa Y.ipt:17 ↔ 0008-10-2012 DIN 125 - A 5.3.ipt:72
- Insert:115: 0008-10-019 Suport Axa Y.ipt:17 ↔ 0008-10-2012 DIN 125 - A 5.3.ipt:75
- [Insert] (-5 mm): 0008-10-2010 M 5 Canal.ipt:76 ↔ 0008-10-2011 DIN 7984 - M5 x 16.ipt:77
- [Insert]: 0008-10-2011 DIN 7984 - M5 x 16.ipt:77 ↔ 0008-10-2012 DIN 125 - A 5.3.ipt:78
- [Insert] (-5 mm): 0008-10-2010 M 5 Canal.ipt:79 ↔ 0008-10-2011 DIN 7984 - M5 x 16.ipt:80
- [Insert]: 0008-10-2011 DIN 7984 - M5 x 16.ipt:80 ↔ 0008-10-2012 DIN 125 - A 5.3.ipt:81
- [Insert] (-5 mm): 0008-10-2010 M 5 Canal.ipt:82 ↔ 0008-10-2011 DIN 7984 - M5 x 16.ipt:83
- [Insert]: 0008-10-2011 DIN 7984 - M5 x 16.ipt:83 ↔ 0008-10-2012 DIN 125 - A 5.3.ipt:84
- [Insert] (-5 mm): 0008-10-2010 M 5 Canal.ipt:85 ↔ 0008-10-2011 DIN 7984 - M5 x 16.ipt:86
- [Insert]: 0008-10-2011 DIN 7984 - M5 x 16.ipt:86 ↔ 0008-10-2012 DIN 125 - A 5.3.ipt:87
- Insert:124: 0008-10-037.ipt:20 ↔ 0008-10-2012 DIN 125 - A 5.3.ipt:87
- Insert:125: 0008-10-037.ipt:20 ↔ 0008-10-2012 DIN 125 - A 5.3.ipt:78
- Insert:126: 0008-10-037.ipt:20 ↔ 0008-10-2012 DIN 125 - A 5.3.ipt:81
- Insert:127: 0008-10-037.ipt:20 ↔ 0008-10-2012 DIN 125 - A 5.3.ipt:84
- [Insert] (-5 mm): 0008-10-2010 M 5 Canal.ipt:88 ↔ 0008-10-2011 DIN 7984 - M5 x 16.ipt:89
- [Insert]: 0008-10-2011 DIN 7984 - M5 x 16.ipt:89 ↔ 0008-10-2012 DIN 125 - A 5.3.ipt:90
- [Insert] (-5 mm): 0008-10-2010 M 5 Canal.ipt:91 ↔ 0008-10-2011 DIN 7984 - M5 x 16.ipt:92
- [Insert]: 0008-10-2011 DIN 7984 - M5 x 16.ipt:92 ↔ 0008-10-2012 DIN 125 - A 5.3.ipt:93
- Insert:132: 0008-10-020 Suport Axa Y.ipt:14 ↔ 0008-10-2012 DIN 125 - A 5.3.ipt:90
- Insert:133: 0008-10-020 Suport Axa Y.ipt:14 ↔ 0008-10-2012 DIN 125 - A 5.3.ipt:93
- Insert:134: 0008-10-2005 DIN 125 - A 3.2.ipt:94 ↔ 0008-10-2006 DIN 7984 - M3 x 16.ipt:95
- [Insert]: 0008-10-2005 DIN 125 - A 3.2.ipt:96 ↔ 0008-10-2006 DIN 7984 - M3 x 16.ipt:97
- [Insert]: 0008-10-2005 DIN 125 - A 3.2.ipt:98 ↔ 0008-10-2006 DIN 7984 - M3 x 16.ipt:99
- [Insert]: 0008-10-2005 DIN 125 - A 3.2.ipt:100 ↔ 0008-10-2006 DIN 7984 - M3 x 16.ipt:101
- Insert:138: 0008-10-048.ipt:24 ↔ 0008-10-2005 DIN 125 - A 3.2.ipt:98
- Insert:139: 0008-10-048.ipt:24 ↔ 0008-10-2005 DIN 125 - A 3.2.ipt:96
- Insert:140: 0008-10-048.ipt:24 ↔ 0008-10-2005 DIN 125 - A 3.2.ipt:100
- Insert:141: 0008-10-048.ipt:24 ↔ 0008-10-2005 DIN 125 - A 3.2.ipt:94
- Insert:142: 0008-10-2000 DIN 6912 - M4 x 25.ipt:102 ↔ 0008-10-2012 DIN 125 - A 5.3.ipt:103
- Insert:143 (-5 mm): 0008-10-2000 DIN 6912 - M4 x 25.ipt:102 ↔ 0008-10-2010 M 5 Canal.ipt:104
- Insert:144: 0008-10-048.ipt:24 ↔ 0008-10-2012 DIN 125 - A 5.3.ipt:103
- [Insert]: 0008-10-2000 DIN 6912 - M4 x 25.ipt:105 ↔ 0008-10-2012 DIN 125 - A 5.3.ipt:106
- [Insert] (-5 mm): 0008-10-2000 DIN 6912 - M4 x 25.ipt:105 ↔ 0008-10-2010 M 5 Canal.ipt:107
- Insert:147: 0008-10-048.ipt:24 ↔ 0008-10-2012 DIN 125 - A 5.3.ipt:106
- [Insert]: 0008-10-2002 DIN 125 - A 4.3.ipt:109 ↔ 0008-10-2001 DIN 934 - M4 x 0.7.ipt:110
- [Insert]: 0008-10-2018 DIN 912 - M4 x 0.7 x 40.ipt:108 ↔ 0008-10-2002 DIN 125 - A 4.3.ipt:111
- [Insert] (2 mm): 0008-10-2018 DIN 912 - M4 x 0.7 x 40.ipt:108 ↔ 0008-10-2001 DIN 934 - M4 x 0.7.ipt:110
- Insert:151: 0008-10-037.ipt:20 ↔ 0008-10-2002 DIN 125 - A 4.3.ipt:111
- [Insert]: 0008-10-2002 DIN 125 - A 4.3.ipt:113 ↔ 0008-10-2001 DIN 934 - M4 x 0.7.ipt:114
- [Insert]: 0008-10-2018 DIN 912 - M4 x 0.7 x 40.ipt:112 ↔ 0008-10-2002 DIN 125 - A 4.3.ipt:115
- [Insert] (2 mm): 0008-10-2018 DIN 912 - M4 x 0.7 x 40.ipt:112 ↔ 0008-10-2001 DIN 934 - M4 x 0.7.ipt:114
- Insert:158: 0008-10-037.ipt:20 ↔ 0008-10-2002 DIN 125 - A 4.3.ipt:115
- Mate:221: 0008-10-037.ipt:20 ↔ 0008-10-1023 Compress Spring11.ipt:160
- Mate:222: 0008-10-2018 DIN 912 - M4 x 0.7 x 40.ipt:112 ↔ 0008-10-1023 Compress Spring11.ipt:160
- Mate:223: 0008-10-01 Sckeleton_Shrinkwrap.ipt:37 ↔ 0008-10-1026 wire chain Y.ipt:43
- Mate:225 (80 mm): 0008-10-01 Sckeleton_Shrinkwrap.ipt:37 ↔ 0008-10-1026 wire chain Y.ipt:43
- Insert:159: 0008-10-2016 DIN 315 - M4.ipt:38 ↔ 0008-10-2024 DIN 7991 - M4  x  35.ipt:39
- Insert:160: 0008-10-018 Suport Heated Bed.ipt:3 ↔ 0008-10-2024 DIN 7991 - M4  x  35.ipt:39
- [Insert]: 0008-10-2016 DIN 315 - M4.ipt:40 ↔ 0008-10-2024 DIN 7991 - M4  x  35.ipt:41
- [Insert]: 0008-10-2016 DIN 315 - M4.ipt:42 ↔ 0008-10-2024 DIN 7991 - M4  x  35.ipt:44
- [Insert]: 0008-10-2016 DIN 315 - M4.ipt:45 ↔ 0008-10-2024 DIN 7991 - M4  x  35.ipt:46
- Insert:164: 0008-10-018 Suport Heated Bed.ipt:3 ↔ 0008-10-2024 DIN 7991 - M4  x  35.ipt:41
- Insert:165: 0008-10-018 Suport Heated Bed.ipt:3 ↔ 0008-10-2024 DIN 7991 - M4  x  35.ipt:44
- Insert:166: 0008-10-018 Suport Heated Bed.ipt:3 ↔ 0008-10-2024 DIN 7991 - M4  x  35.ipt:46
- Mate:226: 0008-10-018 Suport Heated Bed.ipt:3 ↔ 0008-10-1023 Compress Spring11.ipt:163
- Mate:227: 0008-10-2024 DIN 7991 - M4  x  35.ipt:41 ↔ 0008-10-1023 Compress Spring11.ipt:163
- Insert:167: 0008-10-2027 DIN 7984 - M3 x 5.ipt:167 ↔ 0008-10-2005 DIN 125 - A 3.2.ipt:168
- Insert:168: 0008-20-1007 HEATING BED.ipt:35 ↔ 0008-10-2005 DIN 125 - A 3.2.ipt:168
- [Insert]: 0008-10-2027 DIN 7984 - M3 x 5.ipt:169 ↔ 0008-10-2005 DIN 125 - A 3.2.ipt:170
- [Insert]: 0008-10-2027 DIN 7984 - M3 x 5.ipt:171 ↔ 0008-10-2005 DIN 125 - A 3.2.ipt:172
- [Insert]: 0008-10-2027 DIN 7984 - M3 x 5.ipt:173 ↔ 0008-10-2005 DIN 125 - A 3.2.ipt:174
- [Insert]: 0008-10-2027 DIN 7984 - M3 x 5.ipt:175 ↔ 0008-10-2005 DIN 125 - A 3.2.ipt:176
- [Insert]: 0008-10-2027 DIN 7984 - M3 x 5.ipt:177 ↔ 0008-10-2005 DIN 125 - A 3.2.ipt:178
- [Insert]: 0008-10-2027 DIN 7984 - M3 x 5.ipt:179 ↔ 0008-10-2005 DIN 125 - A 3.2.ipt:180
- [Insert]: 0008-10-2027 DIN 7984 - M3 x 5.ipt:181 ↔ 0008-10-2005 DIN 125 - A 3.2.ipt:182
- Insert:176: 0008-20-1007 HEATING BED.ipt:35 ↔ 0008-10-2005 DIN 125 - A 3.2.ipt:170
- Insert:177: 0008-20-1007 HEATING BED.ipt:35 ↔ 0008-10-2005 DIN 125 - A 3.2.ipt:172
- Insert:178: 0008-20-1007 HEATING BED.ipt:35 ↔ 0008-10-2005 DIN 125 - A 3.2.ipt:174
- Insert:179: 0008-20-1007 HEATING BED.ipt:36 ↔ 0008-10-2005 DIN 125 - A 3.2.ipt:182
- Insert:180: 0008-20-1007 HEATING BED.ipt:36 ↔ 0008-10-2005 DIN 125 - A 3.2.ipt:180
- Insert:181: 0008-20-1007 HEATING BED.ipt:36 ↔ 0008-10-2005 DIN 125 - A 3.2.ipt:178
- Insert:182: 0008-20-1007 HEATING BED.ipt:36 ↔ 0008-10-2005 DIN 125 - A 3.2.ipt:176
- Mate:228 (20 mm): 0008-10-1016 SC10UU.ipt:4 ↔ 0008-10-1026 wire chain Y.ipt:43
- Insert:183: 0008-10-020 Suport Axa Y.ipt:13 ↔ SurubM4x25:3
- Insert:184: 0008-10-020 Suport Axa Y.ipt:9 ↔ SurubM4x25:4
- Insert:185: 0008-10-020 Suport Axa Y.ipt:14 ↔ SurubM4x25:5
- Insert:186: 0008-10-052 Suport Axa Y +Senzor.ipt:10 ↔ SurubM4x25:6
- Insert:187: 0008-10-019 Suport Axa Y.ipt:16 ↔ SurubM4x25:7
- Insert:188: 0008-10-019 Suport Axa Y.ipt:17 ↔ SurubM4x25:8
- Insert:190: 0008-10-036.ipt:21 ↔ DIN 7984 M5 x 20:1
- Insert:191: 0008-10-018 Suport Heated Bed.ipt:3 ↔ 0008-10-054 Suport doking.ipt:26
- Mate:229: 0008-10-054 Suport doking.ipt:26 ↔ 0008-10-2017 DIN 7991 - M4x20.ipt:30
## Named parameters: d168_d159 = 0 mm, d169_d160 = 0 mm, d170_d163 = 0 deg, d171_d164 = 0 mm, d172_d165 = 0 mm, d223_d120_d113 = 0 mm, d462_d461 = 0 mm, d482_d472 = -3 mm, d487_d2 = 0 mm, d488_d2 = 0 mm, d489_d2 = 0 mm, d494_d2 = 0 mm, d495_d2 = 0 mm, d496_d2 = 0 mm, d497_d2 = 0 mm, d502_d2 = 0 mm, d503_d2 = 0 mm, d504_d2 = 0 mm, d505_d2 = 0 mm, d510_d2 = 0 mm, d511_d2 = 0 mm, d512_d2 = 0 mm, d513_d2 = 0 mm, d518_d2 = 0 mm, d519_d2 = 0 mm, d520_d2 = 0 mm, d521_d2 = 0 mm, d481_d455 = -5 mm, d482_d456 = 0 mm, d529_d481_d455 = -5 mm, d530_d482_d456 = 0 mm, d531_d481_d455 = -5 mm, d532_d482_d456 = 0 mm, d533_d481_d455 = -5 mm, d534_d482_d456 = 0 mm, d538_d481_d455 = -5 mm, d539_d482_d456 = 0 mm, d540_d481_d455 = -5 mm, d541_d482_d456 = 0 mm, d546_d538_d481_d455 = -5 mm, d547_d539_d482_d456 = 0 mm, d548_d538_d481_d455 = -5 mm, d549_d539_d482_d456 = 0 mm, d550_d538_d481_d455 = -5 mm, d551_d539_d482_d456 = 0 mm, d552_d538_d481_d455 = -5 mm, d553_d539_d482_d456 = 0 mm, d558_d538_d481_d455 = -5 mm, d559_d539_d482_d456 = 0 mm, d560_d538_d481_d455 = -5 mm, d561_d539_d482_d456 = 0 mm, d562_d538_d481_d455 = -5 mm, d563_d539_d482_d456 = 0 mm, d564_d538_d481_d455 = -5 mm, d565_d539_d482_d456 = 0 mm, d570_d538_d481_d455 = -5 mm, d571_d539_d482_d456 = 0 mm, d572_d538_d481_d455 = -5 mm, d573_d539_d482_d456 = 0 mm, d577_d576 = 0 mm, d578_d576 = 0 mm, d579_d576 = 0 mm, d587_d584 = 0 mm, d588_d585 = -5 mm, d755_d558_d539_d533_d477 = 0 mm, d756_d559_d540 = 0 mm, d757_d560_d541 = 2 mm, d599_d755_d558_d539_d533_d477 = 0 mm, d600_d756_d559_d540 = 0 mm, d601_d757_d560_d541 = 2 mm, d616_d614 = 0 mm, d617_d614 = 0 mm, d618_d614 = 0 mm, d630_d628 = 0 mm, d631_d628 = 0 mm, d632_d628 = 0 mm, d633_d628 = 0 mm, d634_d628 = 0 mm, d635_d628 = 0 mm, d636_d628 = 0 mm
